# Autodesk Inventor assembly: kinetic furniture_extension table
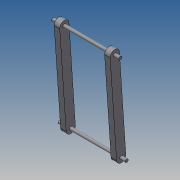
[picture p0: Inventor's stored thumbnail of the model, 180x180]
Saved by Autodesk Inventor 2019 (Build 230136000, 136)
## iProperties
Created: 2021-12-12
Part Number: kinetic furniture_extension table
Document SubType Name: Assembly
Designer: Yongwoo Song_mjkga
Author: Yongwoo Song_mjkga
## Documents named in this file (3)
- C:\Users\Public\Documents\Autodesk\Inventor 2019\Inventor Practice(mjkga)\kinetic furniture_extension table.iam
- X:\Fab-Make-21\211212_mechanism practice\Bar part1.ipt
- C:\Users\Public\Documents\Autodesk\Inventor 2019\woodpipe.ipt
## Components (4 placed, 2 different names)
1. woodpipe:1 — Rigid:3, Rigid:4
2. Bar part1:1 — Rigid:4, Rigid:6
3. Bar part1:2 — Rigid:3, Rigid:5
4. woodpipe:2 — Rigid:5, Rigid:6
## Relationships (4: WeldJoint 4)
- Rigid:3 [WeldJoint] (-18 mm): woodpipe:1 ↔ Bar part1:2
- Rigid:4 [WeldJoint] (-18 mm): woodpipe:1 ↔ Bar part1:1
- Rigid:5 [WeldJoint] (18 mm): Bar part1:2 ↔ woodpipe:2
- Rigid:6 [WeldJoint] (-18 mm): Bar part1:1 ↔ woodpipe:2
